# Autodesk Inventor assembly: Design Training 2_Gearboxes_Exercise 1
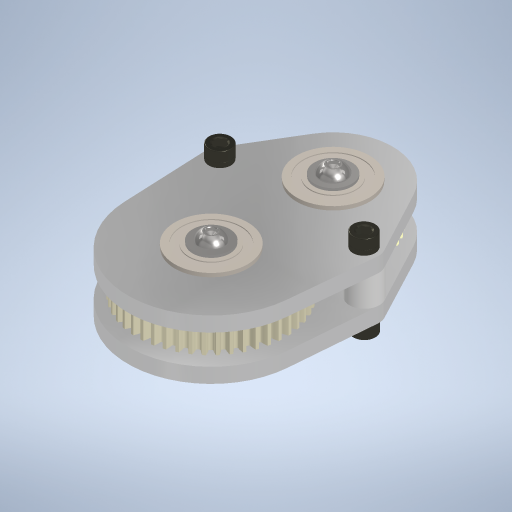
[picture p0: Inventor's stored thumbnail of the model, 512x512]
Saved by Autodesk Inventor 2024 (Build 280153000, 153)
## iProperties
Created: 2024-07-14
Part Number: Design Training 2_Gearboxes_Exercise 1
Document SubType Name: Assembly
Designer: Danielle
Author: Danielle
## Documents named in this file (11)
- C:\Users\micha\OneDrive\Documents\Design Training 2_Gearboxes_Exercise 1.iam
- C:\Users\micha\OneDrive\Documents\BottomPlate.ipt
- C:\Users\micha\OneDrive\Documents\TopPlate.ipt
- C:\Users\micha\Downloads\WCP-0783\WCP-0783.ipt
- C:\Users\micha\Downloads\WCP-0188\WCP-0188.ipt
- C:\Users\micha\Downloads\WCP-0707\WCP-0707.ipt
- C:\Users\micha\OneDrive\Documents\1.123 in. Hex Shaft.ipt
- C:\Users\micha\Downloads\92949A535_18-8 Stainless Steel Button Head Hex Drive Screw\92949A535_18-8 Stainless Steel Button Head Hex Drive Screw.ipt
- C:\Users\micha\Downloads\90107A029_316 Stainless Steel Washer\90107A029_316 Stainless Steel Washer.ipt
- C:\Users\micha\Downloads\WCP-0783\0.5 in long x 0.5 in wide x 0.257 in tap standoff.ipt
- C:\Users\micha\OneDrive\Documents\GitHub\1622-2024-Assignments\COTS Library\Fasteners\Bolts\Socket-Head\0.25-20\COTS_91251A537_Black-Oxide Alloy Steel Socket Head Screw.ipt
## Components (24 placed, 10 different names)
1. BottomPlate:1 — Mate:1, Mate:2, Mate:3, Mate:4, Mate:5, Mate:6, Mate:7, Mate:8, Mate:9, Mate:10, Mate:15, Mate:17, Mate:48, Mate:49, Mate:50, Mate:51
2. TopPlate:1 — Mate:1, Mate:2, Mate:11, Mate:12, Mate:13, Mate:14, Mate:16, Mate:18, Flush:2, Flush:3, Flush:4, Mate:44, Mate:45, Mate:46, Mate:47
3. WCP-0783:1 — Mate:8, Mate:10, Angle:4
4. WCP-0188:1 — Mate:3, Flush:1, Mate:5, Mate:19, Mate:20, Angle:1, Angle:2
5. WCP-0707:1 — Mate:4, Flush:1, Mate:6, Angle:3, Angle:4
6. WCP-0783:2 — Mate:7, Mate:9, Mate:19, Angle:2
7. WCP-0783:3 — Mate:12, Mate:14, Angle:3, Flush:6, Mate:22, Angle:6
8. WCP-0783:4 — Mate:11, Mate:13, Mate:20, Angle:1, Mate:21, Flush:5, Angle:5
9. 0.5 in long x 0.5 in wide x 0.257 in tap standoff:1 — Mate:15, Mate:16
10. 0.5 in long x 0.5 in wide x 0.257 in tap standoff:2 — Mate:17, Mate:18
11. 1.123 in. Hex Shaft:1 — Mate:21, Flush:5, Angle:5, Mate:23, Mate:24, Mate:27, Mate:28, Mate:31, Mate:33, Mate:35, Mate:36, Angle:9, Angle:10
12. 1.123 in. Hex Shaft:2 — Flush:6, Mate:22, Angle:6, Mate:25, Mate:26, Mate:34, Angle:7, Mate:37, Mate:38, Mate:39, Angle:8, Angle:11
13. 92949A535_18-8 Stainless Steel Button Head Hex Drive Screw:1 — Mate:34, Mate:42
14. 90107A029_316 Stainless Steel Washer:1 — Mate:25, Mate:26, Angle:7, Angle:11, Mate:42
15. 92949A535_18-8 Stainless Steel Button Head Hex Drive Screw:2 — Mate:33, Mate:43
16. 90107A029_316 Stainless Steel Washer:3 — Mate:27, Mate:28, Mate:36, Angle:9, Mate:40
17. 92949A535_18-8 Stainless Steel Button Head Hex Drive Screw:4 — Mate:31, Mate:40
18. 90107A029_316 Stainless Steel Washer:4 — Mate:23, Mate:24, Mate:35, Angle:10, Mate:43
19. 90107A029_316 Stainless Steel Washer:5 — Mate:37, Mate:38, Angle:8, Mate:41
20. 92949A535_18-8 Stainless Steel Button Head Hex Drive Screw:5 — Mate:39, Mate:41
21. COTS_91251A537_Black-Oxide Alloy Steel Socket Head Screw:1 — Mate:45, Mate:46
22. COTS_91251A537_Black-Oxide Alloy Steel Socket Head Screw:2 — Mate:44, Mate:47
23. COTS_91251A537_Black-Oxide Alloy Steel Socket Head Screw:3 — Mate:49, Mate:51
24. COTS_91251A537_Black-Oxide Alloy Steel Socket Head Screw:4 — Mate:48, Mate:50
## Relationships (65: Mate 48, Angle 11, Flush 6)
- Mate:1: BottomPlate:1 ↔ TopPlate:1
- Mate:2: BottomPlate:1 ↔ TopPlate:1
- Mate:3: BottomPlate:1 ↔ WCP-0188:1
- Mate:4: BottomPlate:1 ↔ WCP-0707:1
- Flush:1: WCP-0188:1 ↔ WCP-0707:1
- Mate:5: BottomPlate:1 ↔ WCP-0188:1
- Mate:6: BottomPlate:1 ↔ WCP-0707:1
- Mate:7: BottomPlate:1 ↔ WCP-0783:2
- Mate:8: BottomPlate:1 ↔ WCP-0783:1
- Mate:9: BottomPlate:1 ↔ WCP-0783:2
- Mate:10: BottomPlate:1 ↔ WCP-0783:1
- Mate:11: TopPlate:1 ↔ WCP-0783:4
- Mate:12: TopPlate:1 ↔ WCP-0783:3
- Mate:13: TopPlate:1 ↔ WCP-0783:4
- Mate:14: TopPlate:1 ↔ WCP-0783:3
- Mate:15: BottomPlate:1 ↔ 0.5 in long x 0.5 in wide x 0.257 in tap standoff:1
- Mate:16: TopPlate:1 ↔ 0.5 in long x 0.5 in wide x 0.257 in tap standoff:1
- Mate:17: BottomPlate:1 ↔ 0.5 in long x 0.5 in wide x 0.257 in tap standoff:2
- Mate:18: TopPlate:1 ↔ 0.5 in long x 0.5 in wide x 0.257 in tap standoff:2
- Mate:19: WCP-0188:1 ↔ WCP-0783:2
- Mate:20: WCP-0188:1 ↔ WCP-0783:4
- Angle:1 (0 deg): WCP-0188:1 ↔ WCP-0783:4
- Angle:2 (0 deg): WCP-0188:1 ↔ WCP-0783:2
- Angle:3 (0 deg): WCP-0707:1 ↔ WCP-0783:3
- Angle:4 (0 deg): WCP-0783:1 ↔ WCP-0707:1
- Flush:2: TopPlate:1
- Flush:3: TopPlate:1
- Flush:4: TopPlate:1
- Mate:21: WCP-0783:4 ↔ 1.123 in. Hex Shaft:1
- Flush:5: WCP-0783:4 ↔ 1.123 in. Hex Shaft:1
- Flush:6: WCP-0783:3 ↔ 1.123 in. Hex Shaft:2
- Mate:22: WCP-0783:3 ↔ 1.123 in. Hex Shaft:2
- Angle:5 (0 deg): WCP-0783:4 ↔ 1.123 in. Hex Shaft:1
- Angle:6 (0 deg): WCP-0783:3 ↔ 1.123 in. Hex Shaft:2
- Mate:23: 1.123 in. Hex Shaft:1 ↔ 90107A029_316 Stainless Steel Washer:4
- Mate:24: 1.123 in. Hex Shaft:1 ↔ 90107A029_316 Stainless Steel Washer:4
- Mate:25: 1.123 in. Hex Shaft:2 ↔ 90107A029_316 Stainless Steel Washer:1
- Mate:26: 1.123 in. Hex Shaft:2 ↔ 90107A029_316 Stainless Steel Washer:1
- Mate:27: 1.123 in. Hex Shaft:1 ↔ 90107A029_316 Stainless Steel Washer:3
- Mate:28: 1.123 in. Hex Shaft:1 ↔ 90107A029_316 Stainless Steel Washer:3
- Mate:31: 1.123 in. Hex Shaft:1 ↔ 92949A535_18-8 Stainless Steel Button Head Hex Drive Screw:4
- Mate:33: 1.123 in. Hex Shaft:1 ↔ 92949A535_18-8 Stainless Steel Button Head Hex Drive Screw:2
- Mate:34: 1.123 in. Hex Shaft:2 ↔ 92949A535_18-8 Stainless Steel Button Head Hex Drive Screw:1
- Mate:35: 1.123 in. Hex Shaft:1 ↔ 90107A029_316 Stainless Steel Washer:4
- Angle:7 (0 deg): 1.123 in. Hex Shaft:2 ↔ 90107A029_316 Stainless Steel Washer:1
- Mate:36: 1.123 in. Hex Shaft:1 ↔ 90107A029_316 Stainless Steel Washer:3
- Mate:37: 1.123 in. Hex Shaft:2 ↔ 90107A029_316 Stainless Steel Washer:5
- Mate:38: 1.123 in. Hex Shaft:2 ↔ 90107A029_316 Stainless Steel Washer:5
- Mate:39: 1.123 in. Hex Shaft:2 ↔ 92949A535_18-8 Stainless Steel Button Head Hex Drive Screw:5
- Angle:8 (0 deg): 1.123 in. Hex Shaft:2 ↔ 90107A029_316 Stainless Steel Washer:5
- Angle:9 (0 deg): 1.123 in. Hex Shaft:1 ↔ 90107A029_316 Stainless Steel Washer:3
- Angle:10 (0 deg): 1.123 in. Hex Shaft:1 ↔ 90107A029_316 Stainless Steel Washer:4
- Angle:11 (0 deg): 1.123 in. Hex Shaft:2 ↔ 90107A029_316 Stainless Steel Washer:1
- Mate:40: 90107A029_316 Stainless Steel Washer:3 ↔ 92949A535_18-8 Stainless Steel Button Head Hex Drive Screw:4
- Mate:41: 90107A029_316 Stainless Steel Washer:5 ↔ 92949A535_18-8 Stainless Steel Button Head Hex Drive Screw:5
- Mate:42: 92949A535_18-8 Stainless Steel Button Head Hex Drive Screw:1 ↔ 90107A029_316 Stainless Steel Washer:1
- Mate:43: 92949A535_18-8 Stainless Steel Button Head Hex Drive Screw:2 ↔ 90107A029_316 Stainless Steel Washer:4
- Mate:44: TopPlate:1 ↔ COTS_91251A537_Black-Oxide Alloy Steel Socket Head Screw:2
- Mate:45: TopPlate:1 ↔ COTS_91251A537_Black-Oxide Alloy Steel Socket Head Screw:1
- Mate:46: TopPlate:1 ↔ COTS_91251A537_Black-Oxide Alloy Steel Socket Head Screw:1
- Mate:47: TopPlate:1 ↔ COTS_91251A537_Black-Oxide Alloy Steel Socket Head Screw:2
- Mate:48: BottomPlate:1 ↔ COTS_91251A537_Black-Oxide Alloy Steel Socket Head Screw:4
- Mate:49: BottomPlate:1 ↔ COTS_91251A537_Black-Oxide Alloy Steel Socket Head Screw:3
- Mate:50: BottomPlate:1 ↔ COTS_91251A537_Black-Oxide Alloy Steel Socket Head Screw:4
- Mate:51: BottomPlate:1 ↔ COTS_91251A537_Black-Oxide Alloy Steel Socket Head Screw:3
